# Autodesk Inventor assembly: frame
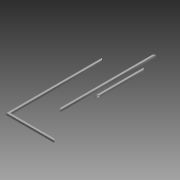
[picture p0: Inventor's stored thumbnail of the model, 180x180]
Saved by Autodesk Inventor 2019 (Build 230136000, 136)
## iProperties
Created: 2019-04-23
Part Number: frame
Document SubType Name: Weldment
Designer: Callum Snowden
Weld Material: Welded Aluminum-6061
Mass: 9459.39 g
Surface Area: 9678.36 cm^2
Volume: 1206 cm^3
Density: 7.84361 g/cm^3
Author: Callum Snowden
## Documents named in this file (4)
- C:\Users\Callum\Documents\GitHub\clasohlsonkart\mechanical\frame\frame.iam
- C:\Users\Callum\Documents\GitHub\clasohlsonkart\mechanical\frame\750mm_box_section.ipt
- C:\Users\Callum\Documents\GitHub\clasohlsonkart\mechanical\frame\1500mm_box_section.ipt
- C:\Users\Callum\Documents\GitHub\clasohlsonkart\mechanical\frame\1500mm_box_section_MIR.ipt
## Components (4 placed, 3 different names)
1. 750mm_box_section:1 — Rigid:1
2. 750mm_box_section:2
3. 1500mm_box_section:1 — Rigid:1
4. 1500mm_box_section_MIR:1
## Relationships (1: WeldJoint 1)
- Rigid:1 [WeldJoint]: 750mm_box_section:1 ↔ 1500mm_box_section:1
